# Autodesk Inventor assembly: дрон сборка
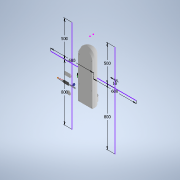
[picture p0: Inventor's stored thumbnail of the model, 180x180]
Saved by Autodesk Inventor 2022.1 (Build 261234000, 234)
## iProperties
Created: 2021-12-25
Part Number: дрон сборка
Document SubType Name: Assembly
Designer: Grigori
Author: Grigori
## Documents named in this file (12)
- C:\Users\Grigo\Desktop\Дрон\Сборка\дрон сборка.iam
- C:\Users\Grigo\Desktop\Дрон\Сборка\корпус.ipt
- C:\Users\Grigo\Desktop\ModularDrone\PartsModels\Ardupilot\APM 2.5 Side Entry Case.ipt
- C:\Users\Grigo\Desktop\ModularDrone\PartsModels\ESC\esc 80A.ipt
- C:\Users\Grigo\Desktop\ModularDrone\PartsModels\GPS\PX4 Neo M8N GPS.ipt
- C:\Users\Grigo\Desktop\ModularDrone\PartsModels\Servo\SG90\SG90 v1.ipt
- C:\Users\Grigo\Desktop\ModularDrone\PartsModels\Telemetry\3D Robotics Radio Telemetry Kit.ipt
- C:\Users\Grigo\Desktop\ModularDrone\PartsModels\Winch\Treuil Yeah racing\Treuil Yeah racing.ipt
- C:\Users\Grigo\Desktop\ModularDrone\PartsModels\Box Battery\Сборка.ipt
- C:\Users\Grigo\Desktop\Дрон\Сборка\Крышка на отсек с батареей.ipt
- C:\Users\Grigo\Documents\Inventor\Content Center Files\R2022\ru-RU\AS 1427(01)\AS 1427 - M3 x 10(3).ipt
- C:\Users\Grigo\Desktop\Дрон\Сборка\Сборка крышка.iam
## Components (18 placed, 11 different names)
1. Корпус:1 — Совмещение:1, Совмещение:2, Совмещение:3, С поворотом:1, С поворотом:2, Совмещение:4, Совмещение:5, Совмещение:6
2. APM 2.5 Side Entry Case:1
3. esc 80A:1
4. PX4 Neo M8N GPS:1
5. SG90 v1:1
6. 3D Robotics Radio Telemetry Kit:1
7. Treuil Yeah racing:1
8. Сборка:1 — Совмещение:1, Совмещение:2, Совмещение:3
9. Крышка на отсек с батареей:1 — С поворотом:1, С поворотом:2, С поворотом:3, С поворотом:4, Жесткий:2, С поворотом:5, Жесткий:3, Жесткий:4, Жесткий:5, Жесткий:6
10. AS 1427 - метрическая M3 x 10:1 — Жесткий:3
11. AS 1427 - метрическая M3 x 10:2 — Жесткий:2
12. AS 1427 - метрическая M3 x 10:3 — С поворотом:4
13. AS 1427 - метрическая M3 x 10:4 — Жесткий:5
14. AS 1427 - метрическая M3 x 10:5 — Жесткий:6
15. AS 1427 - метрическая M3 x 10:6 — С поворотом:5
16. AS 1427 - метрическая M3 x 10:7 — Жесткий:4
17. AS 1427 - метрическая M3 x 10:8 — С поворотом:3
18. Сборка крышка:1 [sub-assembly] — Совмещение:4, Совмещение:5, Совмещение:6
## Relationships (16: Mate 6, RevoluteJoint 5, WeldJoint 5)
- Совмещение:1 [Mate]: Корпус:1 ↔ Сборка:1
- Совмещение:2 [Mate]: Корпус:1 ↔ Сборка:1
- Совмещение:3 [Mate]: Корпус:1 ↔ Сборка:1
- С поворотом:1 [RevoluteJoint]: Корпус:1 ↔ Крышка на отсек с батареей:1
- С поворотом:2 [RevoluteJoint]: Корпус:1 ↔ Крышка на отсек с батареей:1
- С поворотом:3 [RevoluteJoint]: Крышка на отсек с батареей:1 ↔ AS 1427 - метрическая M3 x 10:8
- С поворотом:4 [RevoluteJoint]: Крышка на отсек с батареей:1 ↔ AS 1427 - метрическая M3 x 10:3
- Жесткий:2 [WeldJoint]: Крышка на отсек с батареей:1 ↔ AS 1427 - метрическая M3 x 10:2
- С поворотом:5 [RevoluteJoint]: Крышка на отсек с батареей:1 ↔ AS 1427 - метрическая M3 x 10:6
- Жесткий:3 [WeldJoint]: Крышка на отсек с батареей:1 ↔ AS 1427 - метрическая M3 x 10:1
- Жесткий:4 [WeldJoint]: Крышка на отсек с батареей:1 ↔ AS 1427 - метрическая M3 x 10:7
- Жесткий:5 [WeldJoint]: Крышка на отсек с батареей:1 ↔ AS 1427 - метрическая M3 x 10:4
- Жесткий:6 [WeldJoint]: Крышка на отсек с батареей:1 ↔ AS 1427 - метрическая M3 x 10:5
- Совмещение:4 [Mate]: Корпус:1 ↔ Сборка крышка:1
- Совмещение:5 [Mate]: Корпус:1 ↔ Сборка крышка:1
- Совмещение:6 [Mate]: Корпус:1 ↔ Сборка крышка:1
